# Autodesk Inventor assembly: POM_T5_04
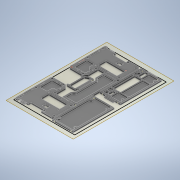
[picture p0: Inventor's stored thumbnail of the model, 180x180]
Saved by Autodesk Inventor 2022.3 (Build 263350000, 350)
## iProperties
Created: 2022-09-28
Part Number: POM_T5_04
Document SubType Name: Assembly
Designer: Masato
Author: Masato
## Documents named in this file (8)
- C:\Users\Masato\Documents\Inventor\Inventor for CIT Brains\SUSTAINA-OP - Cockpit mate\Cam\POM_T5\POM_T5_04.iam
- C:\Users\Masato\Documents\Inventor\Inventor for CIT Brains\SUSTAINA-OP - Cockpit mate\Cam\DisposableBoard.ipt
- C:\Users\Masato\Documents\Inventor\Inventor for CIT Brains\SUSTAINA-OP - Cockpit mate\UpperBody\Cockpit\Cockpit_back_frame.ipt
- C:\Users\Masato\Documents\Inventor\Inventor for CIT Brains\SUSTAINA-OP - Cockpit mate\UpperBody\Cockpit\Cockpit_battery_back_door.ipt
- C:\Users\Masato\Documents\Inventor\Inventor for CIT Brains\SUSTAINA-OP - Cockpit mate\UpperBody\Cockpit\Cockpit_carrier_board_frame.ipt
- C:\Users\Masato\Documents\Inventor\Inventor for CIT Brains\SUSTAINA-OP - Cockpit mate\UpperBody\Cockpit\Cockpit_front_frame.ipt
- C:\Users\Masato\Documents\Inventor\Inventor for CIT Brains\SUSTAINA-OP - Cockpit mate\UpperBody\Cockpit\Cockpit_side_frame.ipt
- C:\Users\Masato\Documents\Inventor\Inventor for CIT Brains\SUSTAINA-OP - Cockpit mate\UpperBody\Cockpit\Cockpit_side_frame_MIR.ipt
## Components (7 placed, 7 different names)
1. DisposableBoard:1 — フラッシュ:1, フラッシュ:2, フラッシュ:3, フラッシュ:4, フラッシュ:5, フラッシュ:6
2. Cockpit_back_frame:1 — メイト:5, フラッシュ:12, フラッシュ:13
3. Cockpit_battery_back_door:1 — メイト:3, メイト:12, フラッシュ:10, メイト:13, メイト:15
4. Cockpit_front_frame:1 — メイト:1, フラッシュ:11, メイト:14, フラッシュ:13
5. Cockpit_side_frame:1 — メイト:7, フラッシュ:5, フラッシュ:6, フラッシュ:9, メイト:12, フラッシュ:10, フラッシュ:11, メイト:14, 正接:1
6. Cockpit_side_frame_MIR:1 — メイト:11, フラッシュ:9, メイト:13, フラッシュ:12
7. Cockpit_carrier_board_frame:2 — メイト:10, メイト:15, 正接:1
## Relationships (22: Flush 11, Mate 10, Tangent 1)
- フラッシュ:1 [Flush]: DisposableBoard:1
- フラッシュ:2 [Flush]: DisposableBoard:1
- フラッシュ:3 [Flush]: DisposableBoard:1
- フラッシュ:4 [Flush]: DisposableBoard:1
- メイト:1 [Mate]: Cockpit_front_frame:1
- メイト:3 [Mate]: Cockpit_battery_back_door:1
- メイト:5 [Mate]: Cockpit_back_frame:1
- メイト:7 [Mate]: Cockpit_side_frame:1
- メイト:10 [Mate]: Cockpit_carrier_board_frame:2
- メイト:11 [Mate]: Cockpit_side_frame_MIR:1
- フラッシュ:5 [Flush] (-2 mm): DisposableBoard:1 ↔ Cockpit_side_frame:1
- フラッシュ:6 [Flush] (2 mm): DisposableBoard:1 ↔ Cockpit_side_frame:1
- フラッシュ:9 [Flush]: Cockpit_side_frame:1 ↔ Cockpit_side_frame_MIR:1
- メイト:12 [Mate] (2.1 mm): Cockpit_battery_back_door:1 ↔ Cockpit_side_frame:1
- フラッシュ:10 [Flush]: Cockpit_battery_back_door:1 ↔ Cockpit_side_frame:1
- メイト:13 [Mate] (2.1 mm): Cockpit_battery_back_door:1 ↔ Cockpit_side_frame_MIR:1
- フラッシュ:11 [Flush]: Cockpit_front_frame:1 ↔ Cockpit_side_frame:1
- フラッシュ:12 [Flush]: Cockpit_back_frame:1 ↔ Cockpit_side_frame_MIR:1
- メイト:14 [Mate] (2.1 mm): Cockpit_front_frame:1 ↔ Cockpit_side_frame:1
- フラッシュ:13 [Flush]: Cockpit_back_frame:1 ↔ Cockpit_front_frame:1
- メイト:15 [Mate] (2.1 mm): Cockpit_battery_back_door:1 ↔ Cockpit_carrier_board_frame:2
- 正接:1 [Tangent] (2.1 mm): Cockpit_side_frame:1 ↔ Cockpit_carrier_board_frame:2
